# Autodesk Inventor assembly: Bauteil 1 Laserhalterung
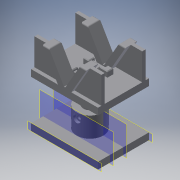
[picture p0: Inventor's stored thumbnail of the model, 180x180]
Saved by Autodesk Inventor 2018.3 (Build 223284000, 284)
## iProperties
Created: 2018-11-29
Part Number: Bauteil 1 Laserhalterung
Material: Generisch
Document SubType Name: Assembly
Designer: pgmadmin
Author: pgmadmin
## Documents named in this file (4)
- C:\Users\alexander.steinhoff\Desktop\Bauteil 1 Laserhalterung.iam
- C:\Users\alexander.steinhoff\Desktop\Laserhalter Mittelteil 29112018.ipt
- C:\Users\alexander.steinhoff\Desktop\Laserhalter Oberteil 29112018.ipt
- C:\Users\alexander.steinhoff\Desktop\Laserhalter Unterteil 29112018.ipt
## Components (3 placed, 3 different names)
1. Laserhalter Mittelteil 29112018:1 — Passend:1, Passend:2, Einfügen:1
2. Laserhalter Oberteil 29112018:1 — Passend:1, Passend:2
3. Laserhalter Unterteil 29112018:1 — Einfügen:1
## Relationships (3: Mate 2, Insert 1)
- Passend:1 [Mate]: Laserhalter Mittelteil 29112018:1 ↔ Laserhalter Oberteil 29112018:1
- Passend:2 [Mate]: Laserhalter Mittelteil 29112018:1 ↔ Laserhalter Oberteil 29112018:1
- Einfügen:1 [Insert] (-5 mm): Laserhalter Mittelteil 29112018:1 ↔ Laserhalter Unterteil 29112018:1
